# Autodesk Inventor assembly: 3dPrinter
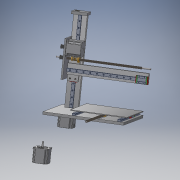
[picture p0: Inventor's stored thumbnail of the model, 180x180]
Saved by Autodesk Inventor 2019 (Build 230136000, 136)
## iProperties
Created: 2018-10-03
Part Number: 3dPrinter
Document SubType Name: Assembly
Designer: LillaHunden
Mass: 5074.53 g
Surface Area: 4765.06 cm^2
Volume: 1725.69 cm^3
Density: 2.94058 g/cm^3
Author: LillaHunden
## Documents named in this file (23)
- C:\Users\LillaHunden\Documents\Inventor\3dprinter\3dPrinter.iam
- C:\Users\LillaHunden\Documents\Inventor\3dprinter\baseplate.ipt
- C:\Users\LillaHunden\Documents\Inventor\3dprinter\Zcolumn.ipt
- C:\Users\LillaHunden\Documents\Inventor\3dprinter\ZcolStiffer.ipt
- C:\Users\LillaHunden\Documents\Inventor\3dprinter\Linear Rials import\Rail Z.ipt
- C:\Users\LillaHunden\Documents\Inventor\3dprinter\Linear Rials import\hotplate.ipt
- C:\Users\LillaHunden\Documents\Inventor\3dprinter\Linear Rials import\MGN block.iam
- C:\Users\LillaHunden\Documents\Inventor\3dprinter\Linear Rials import\Rail Y.ipt
- C:\Users\LillaHunden\Documents\Inventor\3dprinter\Linear Rials import\Xcolum.ipt
- C:\Users\LillaHunden\Documents\Inventor\3dprinter\Linear Rials import\XcolBracket.ipt
- C:\Users\LillaHunden\Documents\Inventor\3dprinter\Linear Rials import\Rail X.ipt
- C:\Users\LillaHunden\Documents\Inventor\3dprinter\3dPrinter\Design Accelerator\Bolted Connection2.iam
- C:\Users\LillaHunden\Documents\Inventor\3dprinter\Linear Rials import\Trapezoidal lead screw tr8x8-4 X.ipt
- C:\Users\LillaHunden\Documents\Inventor\3dprinter\Linear Rials import\Trapezoidal lead screw tr8x8-4 Y.ipt
- C:\Users\LillaHunden\Documents\Inventor\3dprinter\Linear Rials import\Trapezoidal lead screw tr8x8-4 Z.ipt
- C:\Users\LillaHunden\Documents\Inventor\3dprinter\Linear Rials import\TR8_8(P4) Antibacklash Nut w. spring.ipt
- C:\Users\LillaHunden\Documents\Inventor\3dprinter\Linear Rials import\ZnutBracket.ipt
- C:\Users\LillaHunden\Documents\Inventor\3dprinter\3dPrinter\Design Accelerator\Bolted Connection3.iam
- C:\Users\LillaHunden\Documents\Inventor\3dprinter\3dPrinter\Design Accelerator\Bolted Connection4.iam
- C:\Users\LillaHunden\Documents\Inventor\3dprinter\ZBaringBracket.ipt
- C:\Users\LillaHunden\Documents\Inventor\3dprinter\XMotorMount.ipt
- C:\Users\LillaHunden\Documents\Inventor\3dprinter\23hs6403.ipt
- C:\Users\LillaHunden\Documents\Inventor\3dprinter\Pulley import\GT2-20T-9mm\GT2_20T_9mm.ipt
## Components (32 placed, 20 different names)
1. baseplate:1 — Mate:20, Angle:1, Angle:2, Angle:3, Mate:32, Flush:16, Flush:17, Flush:25, Flush:26, Angle:11
2. Zcolumn:1 — Mate:11, Mate:12, Flush:8, Mate:20, Mate:21, Flush:9, Mate:22, Angle:3, Angle:4, Flush:25, Flush:26, Angle:7, Angle:9, Flush:30, Flush:31
3. ZcolStiffer:1 — Mate:11, Mate:12, Flush:8
4. Rail Z:1 — Mate:21, Flush:9, Mate:22, Mate:25, Mate:26
5. hotplate:1 — Mate:23, Mate:24, Flush:10, Flush:12, Angle:1, Angle:2, Flush:17
6. MGN block:1 [sub-assembly] — Mate:25, Angle:4, Mate:26, Flush:13, Mate:27, Flush:14, Flush:18, Flush:19, Flush:22, Mate:38
7. MGN block:2 [sub-assembly] — Flush:13, Mate:27, Flush:14
8. MGN block:3 [sub-assembly] — Mate:23, Flush:11, Symmetry:1, Flush:12, Mate:28, Mate:29
9. MGN block:4 [sub-assembly] — Mate:24, Flush:10, Flush:11, Symmetry:1, Mate:30, Mate:31
10. Rail Y:1 — Mate:30, Mate:31, Flush:15
11. Rail Y:2 — Mate:28, Mate:29, Flush:15, Mate:32, Flush:16, Angle:6
12. Xcolum:1 — Mate:33, Flush:20, Flush:21, Mate:34, Flush:23, Flush:24, Angle:5, Flush:29
13. XcolBracket:1 — Flush:18, Flush:19, Mate:33, Flush:20, Flush:21, Flush:22, Mate:37, Mate:50, Flush:33, Flush:34
14. Rail X:1 — Mate:34, Flush:23, Flush:24, Mate:35, Mate:36
15. MGN block:5 [sub-assembly] — Mate:35, Mate:36
16. Bolted Connection:1 [sub-assembly] — Mate:37, Mate:38
17. Trapezoidal lead screw tr8x8-4 X:1 — Angle:5, Mate:40, Mate:52
18. Trapezoidal lead screw tr8x8-4 Y:1 — Angle:6, Mate:41
19. Trapezoidal lead screw tr8x8-4 Z:1 — Angle:7, Mate:39, Mate:43, Flush:32, Mate:56
20. TR8_8(P4) Antibacklash Nut w. spring:1 — Mate:39, Mate:47, Mate:49
21. TR8_8(P4) Antibacklash Nut w. spring:2 — Mate:40
22. TR8_8(P4) Antibacklash Nut w. spring:3 — Mate:41
23. ZnutBracket:1 — Mate:43, Angle:9, Flush:29, Mate:45, Mate:46, Mate:47, Mate:48
24. Bolted Connection:2 [sub-assembly] — Mate:45, Mate:46
25. Bolted Connection:3 [sub-assembly] — Mate:48, Mate:49
26. ZBaringBracket:1 — Flush:30, Flush:31, Flush:32
27. XMotorMount:1 — Mate:50, Flush:33, Flush:34, Mate:51, Flush:35, Angle:10, Mate:53, Mate:55
28. 23hs6403:1 — Mate:51, Flush:35, Angle:10, Mate:54
29. 23hs6403:2
30. 23hs6403:3 — Mate:56, Angle:11
31. GT2_20T_9mm:1 — Mate:54, Mate:55
32. GT2_20T_9mm:2 — Mate:52, Mate:53
## Relationships (74: Mate 37, Flush 26, Angle 10, Symmetry 1)
- Mate:11: Zcolumn:1 ↔ ZcolStiffer:1
- Mate:12: Zcolumn:1 ↔ ZcolStiffer:1
- Flush:8: Zcolumn:1 ↔ ZcolStiffer:1
- Mate:20 (-5 mm): baseplate:1 ↔ Zcolumn:1
- Mate:21: Zcolumn:1 ↔ Rail Z:1
- Flush:9 (7 mm): Zcolumn:1 ↔ Rail Z:1
- Mate:22: Zcolumn:1 ↔ Rail Z:1
- Mate:23: hotplate:1 ↔ MGN block:3
- Mate:24: hotplate:1 ↔ MGN block:4
- Flush:10 (83 mm): hotplate:1 ↔ MGN block:4
- Flush:11: MGN block:3 ↔ MGN block:4
- Symmetry:1: MGN block:3 ↔ MGN block:4
- Flush:12 (7 mm): hotplate:1 ↔ MGN block:3
- Angle:1 (180 deg): baseplate:1 ↔ hotplate:1
- Angle:2 (90 deg): baseplate:1 ↔ hotplate:1
- Angle:3 (0 deg): baseplate:1 ↔ Zcolumn:1
- Mate:25: Rail Z:1 ↔ MGN block:1
- Angle:4 (0 deg): Zcolumn:1 ↔ MGN block:1
- Mate:26: Rail Z:1 ↔ MGN block:1
- Flush:13: MGN block:1 ↔ MGN block:2
- Mate:27 (7 mm): MGN block:1 ↔ MGN block:2
- Flush:14: MGN block:1 ↔ MGN block:2
- Mate:28: MGN block:3 ↔ Rail Y:2
- Mate:29: MGN block:3 ↔ Rail Y:2
- Mate:30: MGN block:4 ↔ Rail Y:1
- Mate:31: MGN block:4 ↔ Rail Y:1
- Flush:15: Rail Y:1 ↔ Rail Y:2
- Mate:32: baseplate:1 ↔ Rail Y:2
- Flush:16 (4 mm): baseplate:1 ↔ Rail Y:2
- Flush:17 (-2 mm): baseplate:1 ↔ hotplate:1
- Flush:18: MGN block:1 ↔ XcolBracket:1
- Flush:19 (2.5 mm): MGN block:1 ↔ XcolBracket:1
- Mate:33: Xcolum:1 ↔ XcolBracket:1
- Flush:20: Xcolum:1 ↔ XcolBracket:1
- Flush:21 (25 mm): Xcolum:1 ↔ XcolBracket:1
- Flush:22 (-6.5 mm): MGN block:1 ↔ XcolBracket:1
- Mate:34: Xcolum:1 ↔ Rail X:1
- Flush:23: Xcolum:1 ↔ Rail X:1
- Flush:24 (10 mm): Xcolum:1 ↔ Rail X:1
- Mate:35: Rail X:1 ↔ MGN block:5
- Mate:36: Rail X:1 ↔ MGN block:5
- Flush:25 (26 mm): baseplate:1 ↔ Zcolumn:1
- Flush:26 (45 mm): baseplate:1 ↔ Zcolumn:1
- Mate:37: XcolBracket:1 ↔ Bolted Connection:1
- Mate:38: MGN block:1 ↔ Bolted Connection:1
- Angle:5 (0 deg): Xcolum:1 ↔ Trapezoidal lead screw tr8x8-4 X:1
- Angle:6 (0 deg): Rail Y:2 ↔ Trapezoidal lead screw tr8x8-4 Y:1
- Angle:7 (0 deg): Zcolumn:1 ↔ Trapezoidal lead screw tr8x8-4 Z:1
- Mate:39: Trapezoidal lead screw tr8x8-4 Z:1 ↔ TR8_8(P4) Antibacklash Nut w. spring:1
- Mate:40: Trapezoidal lead screw tr8x8-4 X:1 ↔ TR8_8(P4) Antibacklash Nut w. spring:2
- Mate:41: Trapezoidal lead screw tr8x8-4 Y:1 ↔ TR8_8(P4) Antibacklash Nut w. spring:3
- Mate:43: Trapezoidal lead screw tr8x8-4 Z:1 ↔ ZnutBracket:1
- Angle:9 (180 deg): Zcolumn:1 ↔ ZnutBracket:1
- Flush:29: Xcolum:1 ↔ ZnutBracket:1
- Mate:45: ZnutBracket:1 ↔ Bolted Connection:2
- Mate:46: ZnutBracket:1 ↔ Bolted Connection:2
- Mate:47: TR8_8(P4) Antibacklash Nut w. spring:1 ↔ ZnutBracket:1
- Mate:48: ZnutBracket:1 ↔ Bolted Connection:3
- Mate:49: TR8_8(P4) Antibacklash Nut w. spring:1 ↔ Bolted Connection:3
- Flush:30: Zcolumn:1 ↔ ZBaringBracket:1
- Flush:31: Zcolumn:1 ↔ ZBaringBracket:1
- Flush:32: Trapezoidal lead screw tr8x8-4 Z:1 ↔ ZBaringBracket:1
- Mate:50: XcolBracket:1 ↔ XMotorMount:1
- Flush:33: XcolBracket:1 ↔ XMotorMount:1
- Flush:34 (10 mm): XcolBracket:1 ↔ XMotorMount:1
- Mate:51: XMotorMount:1 ↔ 23hs6403:1
- Flush:35 (5 mm): XMotorMount:1 ↔ 23hs6403:1
- Angle:10 (0 deg): XMotorMount:1 ↔ 23hs6403:1
- Mate:52: Trapezoidal lead screw tr8x8-4 X:1 ↔ GT2_20T_9mm:2
- Mate:53 (0.5 mm): XMotorMount:1 ↔ GT2_20T_9mm:2
- Mate:54: 23hs6403:1 ↔ GT2_20T_9mm:1
- Mate:55 (0.5 mm): XMotorMount:1 ↔ GT2_20T_9mm:1
- Mate:56: Trapezoidal lead screw tr8x8-4 Z:1 ↔ 23hs6403:3
- Angle:11 (0 deg): baseplate:1 ↔ 23hs6403:3
